# Autodesk Inventor assembly: axis3
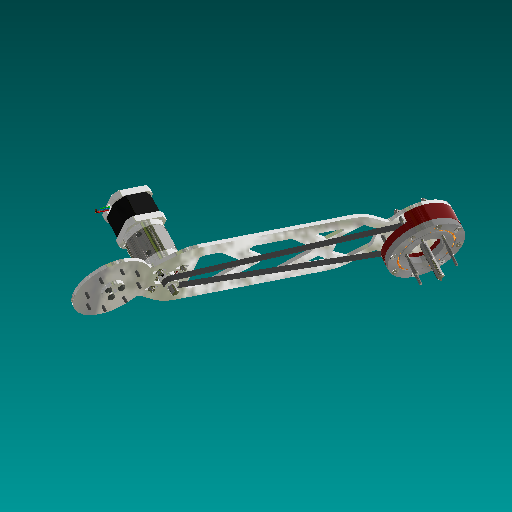
[picture p0: Inventor's stored thumbnail of the model, 512x512]
Saved by Autodesk Inventor 2020.3 (Build 243373000, 373)
## iProperties
Created: 2020-05-24
Part Number: axis3
Document SubType Name: Assembly
Designer: Svend
Author: Svend
## Documents named in this file (25)
- C:\Users\Svend\OneDrive\Documents\GitHub\BeerMinder\3D-model\axis3\axis3.iam
- C:\Users\Svend\OneDrive\Documents\GitHub\BeerMinder\3D-model\subAssembly\Nema17MetGearbox.iam
- C:\Users\Svend\OneDrive\Documents\GitHub\BeerMinder\3D-model\pulleys\GT2 Timing Pulley 20T - 8mm as.ipt
- C:\Users\Svend\OneDrive\Documents\GitHub\BeerMinder\3D-model\pulleys\Tandriem20naar60T-696mm.ipt
- C:\Users\Svend\OneDrive\Documents\GitHub\BeerMinder\3D-model\Base (Axis 1)\spiebaanBevestiging.ipt
- C:\Users\Svend\OneDrive\Documents\GitHub\BeerMinder\3D-model\pulleys\GT2 Timing Pulley 60T - 8mm as.ipt
- C:\Users\Svend\OneDrive\Documents\GitHub\BeerMinder\3D-model\bearings\Ball Bearing 608ZZ.ipt
- C:\Users\Svend\OneDrive\Documents\GitHub\BeerMinder\3D-model\Base (Axis 1)\asArm2.ipt
- C:\Users\Svend\OneDrive\Documents\GitHub\BeerMinder\3D-model\Base (Axis 1)\arm1v2.ipt
- C:\Users\Svend\OneDrive\Documents\GitHub\BeerMinder\3D-model\Base (Axis 1)\60mmspacer.ipt
- C:\Users\Svend\OneDrive\Documents\GitHub\BeerMinder\3D-model\Base (Axis 1)\60mmspacerDicht.ipt
- C:\Users\Svend\OneDrive\Documents\GitHub\BeerMinder\3D-model\bearings\stelring - 8mm.ipt
- C:\Users\Svend\OneDrive\Documents\GitHub\BeerMinder\3D-model\axis4\spacerVoorLager.ipt
- C:\Users\Svend\OneDrive\Documents\Inventor\Content Center Files\R2020\en-US\ISO 4762(2)\ISO 4762 - M3 x 10ISO.ipt
- C:\Users\Svend\OneDrive\Documents\Inventor\Content Center Files\R2020\en-US\ISO 7089\ISO 7089 - 3 - 140 HV(1).ipt
- C:\Users\Svend\OneDrive\Documents\Inventor\Content Center Files\R2020\en-US\ISO 10642(1)\ISO 10642 - M3x12.ipt
- C:\Users\Svend\OneDrive\Documents\Inventor\Content Center Files\R2020\en-US\ISO 4035(2)\ISO 4035 - M3 - ISO.ipt
- C:\Users\Svend\OneDrive\Documents\GitHub\BeerMinder\3D-model\bearings\slew bearing 80 mm\Slew Bearing 80mm.iam
- C:\Users\Svend\OneDrive\Documents\Inventor\Content Center Files\R2020\en-US\ISO 10642(1)\ISO 10642 - M4x35.ipt
- C:\Users\Svend\OneDrive\Documents\Inventor\Content Center Files\R2020\en-US\ISO 7089\ISO 7089 - 4 - 140 HV(1).ipt
- C:\Users\Svend\OneDrive\Documents\Inventor\Content Center Files\R2020\en-US\ISO 4035(2)\ISO 4035 - M4 - ISO.ipt
- C:\Users\Svend\OneDrive\Documents\GitHub\BeerMinder\3D-model\Base (Axis 1)\spiebaanplaatKlein.ipt
- C:\Users\Svend\OneDrive\Documents\Inventor\Content Center Files\R2020\en-US\ISO 7380-1\ISO 7380-1 - M4 x 16.ipt
- C:\Users\Svend\OneDrive\Documents\Inventor\Content Center Files\R2020\en-US\ISO 4762(2)\ISO 4762 - M3 x 30ISO.ipt
- C:\Users\Svend\OneDrive\Documents\Inventor\Content Center Files\R2020\en-US\ISO 7380-1\ISO 7380-1 - M3 x 10.ipt
## Components (75 placed, 24 different names)
1. Nema17MetGearbox:1 [sub-assembly] — Mate:33, Mate:34, Mate:35, Mate:41
2. GT2 Timing Pulley 20T - 8mm as:1
3. Tandriem20naar60T-696mm:1
4. spiebaanBevestiging:1 — Flush:4
5. GT2 Timing Pulley 60T - 8mm as:1
6. Ball Bearing 608ZZ:1
7. asArm2:1
8. arm1v2:1 — Mate:22, Mate:23, Mate:36, Mate:37, Mate:38, Mate:39, Mate:40, Mate:42, Mate:43, Mate:44, Mate:45, Mate:59, Insert:3, Insert:4, Insert:5, Insert:6, Insert:7, Insert:8, Insert:9, Insert:10, Mate:69, Mate:76, Insert:42, Insert:43, Insert:44, Insert:45, Insert:46, Insert:47, Insert:48, Insert:49
9. 60mmspacer:1
10. 60mmspacerDicht:1 — Mate:47, Mate:49, Mate:51, Mate:53
11. stelring - 8mm:1
12. spacerVoorLager:1 — Mate:22, Mate:23, Mate:58, Mate:59, Mate:60
13. spiebaanplaatKlein:1 — Mate:69, Flush:4, Mate:70, Mate:71, Mate:72, Mate:73, Mate:74, Mate:75, Mate:76
14. ISO 7380-1 M3 x 10:1 — Insert:42
15. ISO 7380-1 M3 x 10:2 — Insert:43
16. ISO 7380-1 M3 x 10:3 — Insert:44
17. ISO 7380-1 M3 x 10:4 — Insert:45
18. ISO 7380-1 M3 x 10:5 — Insert:46
19. ISO 7380-1 M3 x 10:6 — Insert:47
20. ISO 7380-1 M3 x 10:7 — Insert:48
21. ISO 7380-1 M3 x 10:8 — Insert:49
22. ISO 7380-1 M4 x 16:1 — Mate:70, Mate:71
23. ISO 7380-1 M4 x 16:3 — Mate:72, Mate:73
24. ISO 7380-1 M4 x 16:2 — Mate:74, Mate:75
25. ISO 4762 M3 x 30:1 — Insert:36
26. ISO 4762 M3 x 30:2 — Insert:37
27. ISO 4762 M3 x 30:3 — Insert:38
28. ISO 4762 M3 x 30:4 — Insert:39
29. ISO 4762 M3 x 30:5 — Insert:40
30. ISO 4762 M3 x 30:6 — Insert:41
31. ISO 4762 M3 x 10:1 — Mate:29, Mate:30, Mate:34
32. ISO 4762 M3 x 10:2 — Mate:25, Mate:26, Mate:35
33. ISO 4762 M3 x 10:3 — Mate:27, Mate:28, Mate:41
34. ISO 4762 M3 x 10:4 — Mate:31, Mate:32, Mate:33
35. ISO 7089 3:1 — Mate:25, Mate:26, Mate:36
36. ISO 7089 3:2 — Mate:27, Mate:28, Mate:37, Mate:38
37. ISO 7089 3:3 — Mate:29, Mate:30, Mate:39
38. ISO 7089 3:4 — Mate:31, Mate:32, Mate:40
39. ISO 10642 M3x12:1 — Mate:42, Mate:48
40. ISO 10642 M3x12:2 — Mate:43, Mate:46, Mate:54
41. ISO 10642 M3x12:3 — Mate:44, Mate:50
42. ISO 10642 M3x12:4 — Mate:45, Mate:52, Mate:56
43. ISO 7089 3:5 — Mate:46, Mate:47, Mate:55
44. ISO 7089 3:6 — Mate:48, Mate:49, Insert:1
45. ISO 7089 3:7 — Mate:50, Mate:51, Insert:2
46. ISO 7089 3:8 — Mate:52, Mate:53, Mate:57
47. ISO 4035 M3:1 — Mate:54, Mate:55
48. ISO 4035 M3:2 — Mate:56, Mate:57
49. ISO 4035 M3:3 — Insert:1
50. ISO 4035 M3:4 — Insert:2
51. Slew Bearing 80mm:1 [sub-assembly] — Mate:58, Mate:60, Mate:61, Mate:62, Mate:63, Mate:64, Mate:65, Mate:66, Mate:67, Mate:68, Insert:36, Insert:37, Insert:38, Insert:39, Insert:40, Insert:41
52. ISO 10642 M4x35:1 — Mate:61
53. ISO 10642 M4x35:2 — Mate:62
54. ISO 10642 M4x35:3 — Mate:63
55. ISO 10642 M4x35:4 — Mate:64
56. ISO 10642 M4x35:5 — Mate:65
57. ISO 10642 M4x35:6 — Mate:66, Mate:77
58. ISO 10642 M4x35:7 — Mate:67
59. ISO 10642 M4x35:8 — Mate:68
60. ISO 7089 4:1 — Insert:3, Insert:32
61. ISO 7089 4:2 — Insert:4, Insert:28
62. ISO 7089 4:3 — Insert:5, Insert:34
63. ISO 7089 4:4 — Insert:6, Insert:30
64. ISO 7089 4:5 — Insert:7, Insert:31
65. ISO 7089 4:6 — Insert:8, Insert:33
66. ISO 7089 4:7 — Insert:9, Insert:35
67. ISO 7089 4:8 — Insert:10, Insert:29
68. ISO 4035 M4:1 — Insert:28
69. ISO 4035 M4:2 — Insert:29
70. ISO 4035 M4:3 — Insert:30
71. ISO 4035 M4:4 — Insert:31
72. ISO 4035 M4:5 — Insert:32, Mate:77
73. ISO 4035 M4:6 — Insert:33
74. ISO 4035 M4:7 — Insert:34
75. ISO 4035 M4:8 — Insert:35
## Relationships (113: Mate 76, Insert 32, Flush 4, Angle 1)
- [Mate]: GT2 Timing Pulley 20T - 8mm as:1 ↔ Tandriem20naar60T-696mm:1
- [Mate]: Tandriem20naar60T-696mm:1 ↔ GT2 Timing Pulley 60T - 8mm as:1
- [Mate] (0.5 mm): Tandriem20naar60T-696mm:1 ↔ GT2 Timing Pulley 60T - 8mm as:1
- [Mate]: GT2 Timing Pulley 60T - 8mm as:1 ↔ Ball Bearing 608ZZ:1
- [Mate]: GT2 Timing Pulley 60T - 8mm as:1 ↔ Ball Bearing 608ZZ:1
- [Mate]: Ball Bearing 608ZZ:1 ↔ asArm2:1
- [Mate]: spiebaanBevestiging:1 ↔ arm1v2:1
- [Flush]: spiebaanBevestiging:1 ↔ arm1v2:1
- [Mate]: Nema17MetGearbox:1 ↔ arm1v2:1
- [Angle] (180 deg): Nema17MetGearbox:1 ↔ arm1v2:1
- [Mate]: Nema17MetGearbox:1 ↔ GT2 Timing Pulley 20T - 8mm as:1
- [Mate] (0.5 mm): GT2 Timing Pulley 20T - 8mm as:1 ↔ Tandriem20naar60T-696mm:1
- [Mate]: Nema17MetGearbox:1 ↔ arm1v2:1
- [Mate]: arm1v2:1 ↔ 60mmspacer:1
- [Mate]: arm1v2:1 ↔ 60mmspacer:1
- [Mate]: arm1v2:1 ↔ 60mmspacer:1
- [Flush]: Ball Bearing 608ZZ:1 ↔ 60mmspacer:1
- [Mate]: 60mmspacer:1 ↔ 60mmspacerDicht:1
- [Mate]: 60mmspacer:1 ↔ 60mmspacerDicht:1
- [Mate]: 60mmspacer:1 ↔ 60mmspacerDicht:1
- [Mate]: asArm2:1 ↔ stelring - 8mm:1
- [Mate]: 60mmspacerDicht:1 ↔ stelring - 8mm:1
- [Flush]: asArm2:1 ↔ stelring - 8mm:1
- [Mate]: arm1v2:1 ↔ stelring - 8mm:1
- [Mate]: spiebaanBevestiging:1 ↔ arm1v2:1
- Mate:22: arm1v2:1 ↔ spacerVoorLager:1
- Mate:23: arm1v2:1 ↔ spacerVoorLager:1
- Mate:25: ISO 4762 M3 x 10:2 ↔ ISO 7089 3:1
- Mate:26: ISO 4762 M3 x 10:2 ↔ ISO 7089 3:1
- Mate:27: ISO 4762 M3 x 10:3 ↔ ISO 7089 3:2
- Mate:28: ISO 4762 M3 x 10:3 ↔ ISO 7089 3:2
- Mate:29: ISO 4762 M3 x 10:1 ↔ ISO 7089 3:3
- Mate:30: ISO 4762 M3 x 10:1 ↔ ISO 7089 3:3
- Mate:31: ISO 4762 M3 x 10:4 ↔ ISO 7089 3:4
- Mate:32: ISO 4762 M3 x 10:4 ↔ ISO 7089 3:4
- Mate:33: Nema17MetGearbox:1 ↔ ISO 4762 M3 x 10:4
- Mate:34: Nema17MetGearbox:1 ↔ ISO 4762 M3 x 10:1
- Mate:35: Nema17MetGearbox:1 ↔ ISO 4762 M3 x 10:2
- Mate:36: arm1v2:1 ↔ ISO 7089 3:1
- Mate:37: arm1v2:1 ↔ ISO 7089 3:2
- Mate:38: arm1v2:1 ↔ ISO 7089 3:2
- Mate:39: arm1v2:1 ↔ ISO 7089 3:3
- Mate:40: arm1v2:1 ↔ ISO 7089 3:4
- Mate:41: Nema17MetGearbox:1 ↔ ISO 4762 M3 x 10:3
- Mate:42: arm1v2:1 ↔ ISO 10642 M3x12:1
- Mate:43: arm1v2:1 ↔ ISO 10642 M3x12:2
- Mate:44: arm1v2:1 ↔ ISO 10642 M3x12:3
- Mate:45: arm1v2:1 ↔ ISO 10642 M3x12:4
- Mate:46: ISO 10642 M3x12:2 ↔ ISO 7089 3:5
- Mate:47: 60mmspacerDicht:1 ↔ ISO 7089 3:5
- Mate:48: ISO 10642 M3x12:1 ↔ ISO 7089 3:6
- Mate:49: 60mmspacerDicht:1 ↔ ISO 7089 3:6
- Mate:50: ISO 10642 M3x12:3 ↔ ISO 7089 3:7
- Mate:51: 60mmspacerDicht:1 ↔ ISO 7089 3:7
- Mate:52: ISO 10642 M3x12:4 ↔ ISO 7089 3:8
- Mate:53: 60mmspacerDicht:1 ↔ ISO 7089 3:8
- Mate:54: ISO 10642 M3x12:2 ↔ ISO 4035 M3:1
- Mate:55: ISO 7089 3:5 ↔ ISO 4035 M3:1
- Mate:56: ISO 10642 M3x12:4 ↔ ISO 4035 M3:2
- Mate:57: ISO 7089 3:8 ↔ ISO 4035 M3:2
- Insert:1: ISO 7089 3:6 ↔ ISO 4035 M3:3
- Insert:2: ISO 7089 3:7 ↔ ISO 4035 M3:4
- Mate:58: spacerVoorLager:1 ↔ Slew Bearing 80mm:1
- Mate:59: arm1v2:1 ↔ spacerVoorLager:1
- Mate:60: spacerVoorLager:1 ↔ Slew Bearing 80mm:1
- Mate:61: Slew Bearing 80mm:1 ↔ ISO 10642 M4x35:1
- Mate:62: Slew Bearing 80mm:1 ↔ ISO 10642 M4x35:2
- Mate:63: Slew Bearing 80mm:1 ↔ ISO 10642 M4x35:3
- Mate:64: Slew Bearing 80mm:1 ↔ ISO 10642 M4x35:4
- Mate:65: Slew Bearing 80mm:1 ↔ ISO 10642 M4x35:5
- Mate:66: Slew Bearing 80mm:1 ↔ ISO 10642 M4x35:6
- Mate:67: Slew Bearing 80mm:1 ↔ ISO 10642 M4x35:7
- Mate:68: Slew Bearing 80mm:1 ↔ ISO 10642 M4x35:8
- Insert:3: arm1v2:1 ↔ ISO 7089 4:1
- Insert:4: arm1v2:1 ↔ ISO 7089 4:2
- Insert:5: arm1v2:1 ↔ ISO 7089 4:3
- Insert:6: arm1v2:1 ↔ ISO 7089 4:4
- Insert:7: arm1v2:1 ↔ ISO 7089 4:5
- Insert:8: arm1v2:1 ↔ ISO 7089 4:6
- Insert:9: arm1v2:1 ↔ ISO 7089 4:7
- Insert:10: arm1v2:1 ↔ ISO 7089 4:8
- Insert:28: ISO 7089 4:2 ↔ ISO 4035 M4:1
- Insert:29: ISO 7089 4:8 ↔ ISO 4035 M4:2
- Insert:30: ISO 7089 4:4 ↔ ISO 4035 M4:3
- Insert:31: ISO 7089 4:5 ↔ ISO 4035 M4:4
- Insert:32: ISO 7089 4:1 ↔ ISO 4035 M4:5
- Insert:33: ISO 7089 4:6 ↔ ISO 4035 M4:6
- Insert:34: ISO 7089 4:3 ↔ ISO 4035 M4:7
- Insert:35: ISO 7089 4:7 ↔ ISO 4035 M4:8
- Mate:69: arm1v2:1 ↔ spiebaanplaatKlein:1
- Flush:4: spiebaanBevestiging:1 ↔ spiebaanplaatKlein:1
- Mate:70: spiebaanplaatKlein:1 ↔ ISO 7380-1 M4 x 16:1
- Mate:71: spiebaanplaatKlein:1 ↔ ISO 7380-1 M4 x 16:1
- Mate:72: spiebaanplaatKlein:1 ↔ ISO 7380-1 M4 x 16:3
- Mate:73: spiebaanplaatKlein:1 ↔ ISO 7380-1 M4 x 16:3
- Mate:74: spiebaanplaatKlein:1 ↔ ISO 7380-1 M4 x 16:2
- Mate:75: spiebaanplaatKlein:1 ↔ ISO 7380-1 M4 x 16:2
- Mate:76: arm1v2:1 ↔ spiebaanplaatKlein:1
- Mate:77: ISO 10642 M4x35:6 ↔ ISO 4035 M4:5
- Insert:36: ISO 4762 M3 x 30:1 ↔ Slew Bearing 80mm:1
- Insert:37: ISO 4762 M3 x 30:2 ↔ Slew Bearing 80mm:1
- Insert:38: ISO 4762 M3 x 30:3 ↔ Slew Bearing 80mm:1
- Insert:39: ISO 4762 M3 x 30:4 ↔ Slew Bearing 80mm:1
- Insert:40: ISO 4762 M3 x 30:5 ↔ Slew Bearing 80mm:1
- Insert:41: ISO 4762 M3 x 30:6 ↔ Slew Bearing 80mm:1
- Insert:42: arm1v2:1 ↔ ISO 7380-1 M3 x 10:1
- Insert:43: arm1v2:1 ↔ ISO 7380-1 M3 x 10:2
- Insert:44: arm1v2:1 ↔ ISO 7380-1 M3 x 10:3
- Insert:45: arm1v2:1 ↔ ISO 7380-1 M3 x 10:4
- Insert:46: arm1v2:1 ↔ ISO 7380-1 M3 x 10:5
- Insert:47: arm1v2:1 ↔ ISO 7380-1 M3 x 10:6
- Insert:48: arm1v2:1 ↔ ISO 7380-1 M3 x 10:7
- Insert:49: arm1v2:1 ↔ ISO 7380-1 M3 x 10:8
